# Autodesk Inventor assembly: LeftMotorCover
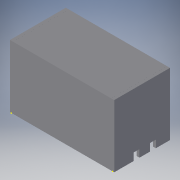
[picture p0: Inventor's stored thumbnail of the model, 180x180]
Saved by Autodesk Inventor 2016 (Build 200138000, 138)
## iProperties
Created: 2016-05-26
Part Number: LeftMotorCover
Document SubType Name: Assembly
Designer: cutrones
Author: cutrones
## Documents named in this file (5)
- C:\Users\cutrones\Desktop\MotionBase\CAD\MotionBaseCAD\MotorCovers\LeftCover\LeftMotorCover.iam
- C:\Users\cutrones\Desktop\MotionBase\CAD\MotionBaseCAD\MotorCovers\LeftCover\InsideWall.ipt
- C:\Users\cutrones\Desktop\MotionBase\CAD\MotionBaseCAD\MotorCovers\LeftCover\OutsideWall.ipt
- C:\Users\cutrones\Desktop\MotionBase\CAD\MotionBaseCAD\MotorCovers\LeftCover\TopWall.ipt
- C:\Users\cutrones\Desktop\MotionBase\CAD\MotionBaseCAD\MotorCovers\LeftCover\SideWall.ipt
## Components (5 placed, 4 different names)
1. InsideWall:1 — Flush:1, Flush:2, Mate:1, Flush:3, Flush:4
2. OutsideWall:1 — Mate:2, Flush:5, Flush:6, Flush:7, Flush:9
3. TopWall:1 — Mate:1, Flush:3, Flush:4, Mate:2, Flush:5, Flush:6, Mate:3, Flush:8, Mate:4, Flush:10
4. SideWall:1 — Flush:9, Mate:4, Flush:10
5. SideWall:2 — Mate:3, Flush:7, Flush:8
## Relationships (14: Flush 10, Mate 4)
- Flush:1: InsideWall:1
- Flush:2: InsideWall:1
- Mate:1: InsideWall:1 ↔ TopWall:1
- Flush:3: InsideWall:1 ↔ TopWall:1
- Flush:4: InsideWall:1 ↔ TopWall:1
- Mate:2: OutsideWall:1 ↔ TopWall:1
- Flush:5: OutsideWall:1 ↔ TopWall:1
- Flush:6: OutsideWall:1 ↔ TopWall:1
- Mate:3: TopWall:1 ↔ SideWall:2
- Flush:7: OutsideWall:1 ↔ SideWall:2
- Flush:8: TopWall:1 ↔ SideWall:2
- Flush:9: OutsideWall:1 ↔ SideWall:1
- Mate:4: TopWall:1 ↔ SideWall:1
- Flush:10: TopWall:1 ↔ SideWall:1
